# Autodesk Inventor assembly: Link3
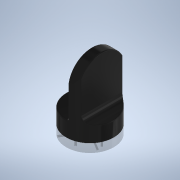
[picture p0: Inventor's stored thumbnail of the model, 180x180]
Saved by Autodesk Inventor 2022 (Build 260153000, 153)
## iProperties
Created: 2022-04-02
Part Number: Link3
Document SubType Name: Assembly
Designer: DDeGo
Author: DDeGo
## Documents named in this file (10)
- C:\Users\DDeGo\Documents\Drew\Projects\OS-ARM\cad\FirstDraft\Link3.iam
- C:\Users\DDeGo\Documents\Drew\Projects\OS-ARM\cad\FirstDraft\Link3.ipt
- C:\Users\DDeGo\Documents\Drew\Projects\OS-ARM\cad\FirstDraft\Wrist.ipt
- C:\Users\DDeGo\Documents\Drew\Projects\OS-ARM\cad\OTS\Electronics\Nema 17 22mm.ipt
- C:\Users\DDeGo\Documents\Drew\Projects\OS-ARM\cad\OTS\Other\GT2Pulley_20T_8mm_noTop.ipt
- C:\Users\DDeGo\Documents\Drew\Projects\OS-ARM\cad\OTS\Thrust Bearings\AXK6085 thrust bearing.ipt
- C:\Users\DDeGo\Documents\Drew\Projects\OS-ARM\cad\FirstDraft\WristMotorPlate.ipt
- C:\Users\DDeGo\Documents\Drew\Projects\OS-ARM\cad\OTS\Other\GT2Pulley_20T_5mm_noTop.ipt
- C:\Users\DDeGo\Documents\Drew\Projects\OS-ARM\cad\OTS\Radial Bearings\685 bearing.ipt
- C:\Users\DDeGo\Documents\Drew\Projects\OS-ARM\cad\FirstDraft\Wrist_planetary.ipt
## Components (9 placed, 9 different names)
1. Link3:1 — Mate:3, Mate:4, Mate:15, Mate:16
2. Wrist:1 — Mate:1, Mate:5, Mate:13, Mate:14
3. Nema 17 22mm:1 — Mate:7, Mate:8, Mate:9, Mate:17, Mate:18
4. GT2Pulley_20T_8mm_noTop:1 — Mate:1, Mate:14
5. AXK6085 thrust bearing:1 — Mate:3, Mate:4, Mate:5, Mate:10, Mate:13, Mate:22
6. WristMotorPlate:1 — Mate:7, Mate:8, Mate:9, Mate:10, Mate:15, Mate:16
7. GT2Pulley_20T_5mm_noTop:1 — Mate:17, Mate:19
8. 685 bearing:1 — Mate:18, Mate:19, Mate:20, Mate:21
9. Wrist_planetary:1 — Mate:20, Mate:21, Mate:22
## Relationships (18: Mate 18)
- Mate:1: Wrist:1 ↔ GT2Pulley_20T_8mm_noTop:1
- Mate:3: Link3:1 ↔ AXK6085 thrust bearing:1
- Mate:4: Link3:1 ↔ AXK6085 thrust bearing:1
- Mate:5: Wrist:1 ↔ AXK6085 thrust bearing:1
- Mate:7: Nema 17 22mm:1 ↔ WristMotorPlate:1
- Mate:8: Nema 17 22mm:1 ↔ WristMotorPlate:1
- Mate:9: Nema 17 22mm:1 ↔ WristMotorPlate:1
- Mate:10: AXK6085 thrust bearing:1 ↔ WristMotorPlate:1
- Mate:13: Wrist:1 ↔ AXK6085 thrust bearing:1
- Mate:14: Wrist:1 ↔ GT2Pulley_20T_8mm_noTop:1
- Mate:15: Link3:1 ↔ WristMotorPlate:1
- Mate:16: Link3:1 ↔ WristMotorPlate:1
- Mate:17: Nema 17 22mm:1 ↔ GT2Pulley_20T_5mm_noTop:1
- Mate:18: Nema 17 22mm:1 ↔ 685 bearing:1
- Mate:19 (0.5 mm): GT2Pulley_20T_5mm_noTop:1 ↔ 685 bearing:1
- Mate:20: 685 bearing:1 ↔ Wrist_planetary:1
- Mate:21: 685 bearing:1 ↔ Wrist_planetary:1
- Mate:22: AXK6085 thrust bearing:1 ↔ Wrist_planetary:1
